# Autodesk Inventor assembly: ADSK-MH-10031
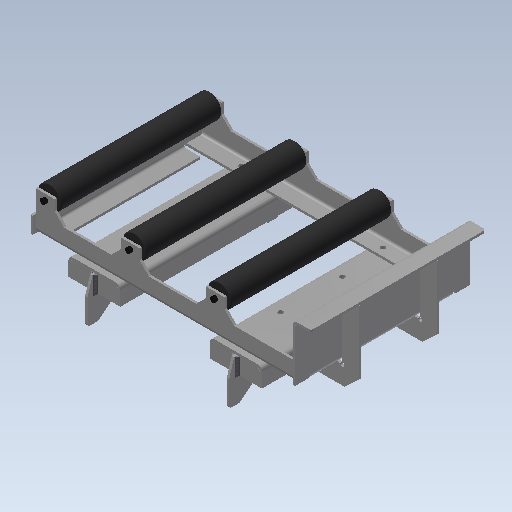
[picture p0: Inventor's stored thumbnail of the model, 512x512]
Saved by Autodesk Inventor 2020.2 (Build 242310000, 310)
## iProperties
Created: 2013-08-01
Part Number: ADSK-MH-10031
Document SubType Name: Assembly
Designer: Demir Ali
Description: Discharge Platform Roller Assembly
Engineer: Demir Ali
Checked By: Demir Ali
Company: Autodesk Ltd
Author: Demir Ali
Keywords: Roller Conveyor
Revision Number: A
## Documents named in this file (9)
- C:\Users\peter\source\repos\InventorDA-FLC\Dataset\Discharge Conveyor\ADSK-MH-10031.iam
- C:\Users\peter\source\repos\InventorDA-FLC\Dataset\Discharge Conveyor\ADSK-MH-10048.ipt
- C:\Users\peter\source\repos\InventorDA-FLC\Dataset\Discharge Conveyor\ADSK-MH-10047.ipt
- C:\Users\peter\source\repos\InventorDA-FLC\Dataset\Discharge Conveyor\ADSK-MH-10038.ipt
- C:\Users\peter\source\repos\InventorDA-FLC\Dataset\Discharge Conveyor\ADSK-MH-10046.iam
- C:\Users\peter\source\repos\InventorDA-FLC\Dataset\Discharge Conveyor\ADSK-MH-10049.iam
- C:\Users\peter\source\repos\InventorDA-FLC\Dataset\Discharge Conveyor\ADSK-MH-10032.ipt
- C:\Users\peter\source\repos\InventorDA-FLC\Dataset\Discharge Conveyor\ADSK-MH-10035.ipt
- C:\Users\peter\source\repos\InventorDA-FLC\Dataset\Discharge Conveyor\ADSK-MH-10036.ipt
## Components (15 placed, 10 different names)
1. Transfer Front — Flush:10, Flush:12, Flush:16, Mate:11
2. Transfer Backplate — Flush:11, Flush:12, Mate:10
3. ADSK-MH-10038:1
4. ADSK-MH-10038:2
5. ADSK-MH-10035:1 — Rigid:3, Flush:14, Flush:15, Mate:10, Mate:11, Mate:12
6. ADSK-MH-10036:1 — Flush:14, Flush:15, Mate:9
7. ADSK-MH-10046:4 [sub-assembly] — Rigid:2
8. Transfer Base — Rigid:1, Rigid:2, Flush:10, Flush:11, Rigid:3, Mate:9, Flush:16, Mate:13
9. ADSK-MH-10046:3 [sub-assembly] — Rigid:1
10. ADSK-MH-10046:5 [sub-assembly]
11. ADSK-MH-10032:2
12. ADSK-MH-10046:6 [sub-assembly]
13. Transfer Roller assem [sub-assembly] — Mate:12, Mate:13
14. ADSK-MH-10049:2 [sub-assembly]
15. ADSK-MH-10049:3 [sub-assembly]
## Component patterns: (2 elements, first: ADSK-MH-10046:4 + Transfer Base + ADSK-MH-10046:3), (3 elements, first: Transfer Roller assem)
## Relationships (20: Mate 9, Flush 8, WeldJoint 3)
- [Mate]: Transfer Backplate ↔ ADSK-MH-10038:1
- [Mate]: Transfer Backplate ↔ ADSK-MH-10038:1
- [Flush] (100 mm): Transfer Backplate ↔ ADSK-MH-10038:1
- [Mate]: Transfer Backplate ↔ ADSK-MH-10038:2
- [Mate]: Transfer Backplate ↔ ADSK-MH-10038:2
- [Flush] (-100 mm): Transfer Backplate ↔ ADSK-MH-10038:2
- Rigid:1 [WeldJoint]: Transfer Base ↔ ADSK-MH-10046:3
- Rigid:2 [WeldJoint]: ADSK-MH-10046:4 ↔ Transfer Base
- Flush:10: Transfer Front ↔ Transfer Base
- Flush:11: Transfer Backplate ↔ Transfer Base
- Flush:12: Transfer Front ↔ Transfer Backplate
- Rigid:3 [WeldJoint]: ADSK-MH-10035:1 ↔ Transfer Base
- Flush:14: ADSK-MH-10035:1 ↔ ADSK-MH-10036:1
- Flush:15: ADSK-MH-10035:1 ↔ ADSK-MH-10036:1
- Mate:9: ADSK-MH-10036:1 ↔ Transfer Base
- Flush:16: Transfer Front ↔ Transfer Base
- Mate:10: Transfer Backplate ↔ ADSK-MH-10035:1
- Mate:11: Transfer Front ↔ ADSK-MH-10035:1
- Mate:12: ADSK-MH-10035:1 ↔ Transfer Roller assem
- Mate:13: Transfer Base ↔ Transfer Roller assem
